# Autodesk Inventor assembly: Ensamble bomba
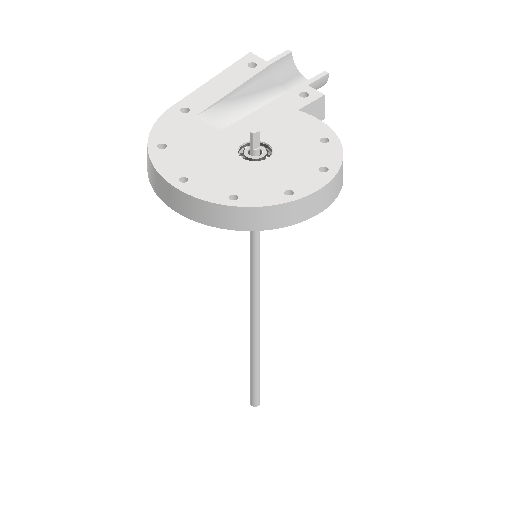
[picture p0: Inventor's stored thumbnail of the model, 512x512]
Saved by Autodesk Inventor 2025.2 (Build 292293000, 293)
## iProperties
Created: 2025-11-12
Part Number: Ensamble bomba
Document SubType Name: Assembly
Designer: juanm
Author: juanm
## Documents named in this file (6)
- C:\Users\nicoa\Documents\GitHub\Proyecto-Turbo\Modelos\Ensamble bomba.iam
- C:\Users\nicoa\Documents\GitHub\Proyecto-Turbo\Modelos\Rodete_4000RPM_2LS.ipt
- C:\Users\nicoa\Documents\GitHub\Proyecto-Turbo\Modelos\Base voluta.ipt
- C:\Users\nicoa\Documents\GitHub\Proyecto-Turbo\Modelos\Tapa voluta.ipt
- C:\Users\nicoa\Documents\GitHub\Proyecto-Turbo\Modelos\Eje 5mm.ipt
- C:\Users\nicoa\Documents\Inventor\Content Center Files\R2025\en-US\BS 290 SKF(29)\BS 290 SKF - SKF 627-2RS1.ipt
## Components (5 placed, 5 different names)
1. Rodete_4000RPM_2LS:1 — Insert:1, Rigid:1
2. Base voluta:1 — Insert:1, Flush:1, Mate:1, Flush:2, Rigid:2
3. Tapa voluta:1 — Flush:1, Mate:1, Flush:2
4. Eje 5mm:1 — Rigid:1
5. BS 290 SKF- with two RS1 seals SKF 627-2RS1:1 — Rigid:2
## Relationships (6: Flush 2, WeldJoint 2, Insert 1, Mate 1)
- Insert:1 (0.5 mm): Rodete_4000RPM_2LS:1 ↔ Base voluta:1
- Flush:1: Base voluta:1 ↔ Tapa voluta:1
- Mate:1: Base voluta:1 ↔ Tapa voluta:1
- Flush:2: Base voluta:1 ↔ Tapa voluta:1
- Rigid:1 [WeldJoint]: Rodete_4000RPM_2LS:1 ↔ Eje 5mm:1
- Rigid:2 [WeldJoint]: Base voluta:1 ↔ BS 290 SKF- with two RS1 seals SKF 627-2RS1:1
